# Autodesk Inventor assembly: encoder
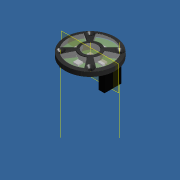
[picture p0: Inventor's stored thumbnail of the model, 180x180]
Saved by Autodesk Inventor 2016 (Build 200138000, 138)
## iProperties
Created: 2015-01-07
Part Number: encoder
Document SubType Name: Assembly
Designer: 4ndreas
Mass: 14.0877 g
Surface Area: 138.088 cm^2
Volume: 13.0717 cm^3
Density: 1.07772 g/cm^3
Author: 4ndreas
## Documents named in this file (4)
- C:\Users\4ndreas\Documents\Inventor\RobotARM v2\v2\encoder.iam
- C:\Users\4ndreas\Documents\Inventor\RobotARM v2\v2\encoder.ipt
- C:\Users\4ndreas\Documents\Inventor\RobotARM v2\v2\encoder_kappe.ipt
- C:\Users\4ndreas\Documents\Inventor\RobotARM v2\v2\encoder_kappe_clear.ipt
## Components (3 placed, 3 different names)
1. encoder:1 — Passend:1, Passend:2, Winkel:1
2. encoder_kappe:1 — Passend:1, Passend:2
3. encoder_kappe_clear:1
## Relationships (4: Mate 3, Angle 1)
- Passend:1 [Mate]: encoder:1 ↔ encoder_kappe:1
- Passend:2 [Mate]: encoder:1 ↔ encoder_kappe:1
- Passend:3 [Mate]
- Winkel:1 [Angle] (90 deg): encoder:1
